# Autodesk Inventor assembly: u_g_Hoehenverstellung_Seiten
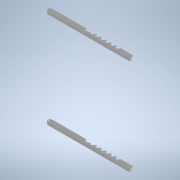
[picture p0: Inventor's stored thumbnail of the model, 180x180]
Saved by Autodesk Inventor 2020.3 (Build 243373000, 373)
## iProperties
Created: 2020-10-05
Part Number: u_g_Hoehenverstellung_Seiten
Document SubType Name: Assembly
Designer: Mara
Author: Mara
## Documents named in this file (3)
- C:\Users\Mara\Masterarbeit_CAD\Rampe\u_g_Hoehenverstellung_Seiten.iam
- C:\Users\Mara\Masterarbeit_CAD\Rampe\u_g_Hoehenverstellung_Seiten.ipt
- C:\Users\Mara\Masterarbeit_CAD\Rampe\u_g_Hoehenverstellung_Seiten_MIR.ipt
## Components (2 placed, 2 different names)
1. u_g_Hoehenverstellung_Seiten:2 — Mate:1, Tangent:1
2. u_g_Hoehenverstellung_Seiten_MIR:1 — Mate:1, Tangent:1
## Relationships (2: Mate 1, Tangent 1)
- Mate:1 (666 mm): u_g_Hoehenverstellung_Seiten:2 ↔ u_g_Hoehenverstellung_Seiten_MIR:1
- Tangent:1: u_g_Hoehenverstellung_Seiten:2 ↔ u_g_Hoehenverstellung_Seiten_MIR:1
